# Autodesk Inventor assembly: Transmission
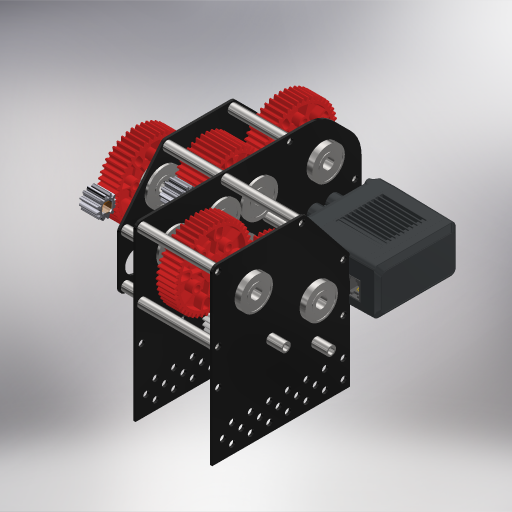
[picture p0: Inventor's stored thumbnail of the model, 512x512]
Saved by Autodesk Inventor 2024 (Build 280153000, 153)
## iProperties
Created: 2023-09-09
Part Number: Transmission
Document SubType Name: Assembly
Designer: aaron
Author: aaron
## Documents named in this file (14)
- C:\Users\aaron\Documents\Inventor\TritonRobotics\library\Stock Material\Plates\POM\Transmision\Transmission.iam
- C:\Users\aaron\Documents\Inventor\TritonRobotics\library\Stock Material\Plates\POM\Transmision\MainLayer.ipt
- C:\Users\aaron\Documents\Inventor\TritonRobotics\library\Stock Material\Plates\POM\Transmision\BottomLayer.ipt
- C:\Users\aaron\Documents\Inventor\TritonRobotics\library\Stock Material\Plates\POM\Transmision\Top Layer.ipt
- C:\Users\aaron\Documents\Inventor\TritonRobotics\library\VEX Library\Structure\Metal Spacers\1.0 1-2 od.ipt
- C:\Users\aaron\Documents\Inventor\TritonRobotics\library\VEX Library\Structure\Metal Spacers\0.25 1-2 od.ipt
- C:\Users\aaron\Documents\Inventor\TritonRobotics\library\VEX Library\Motion\HS Shaft\bearing.ipt
- C:\Users\aaron\Documents\Inventor\TritonRobotics\library\VEX Library\Subsystems\PTOS\PTO .5 v1.1.iam
- C:\Users\aaron\Documents\Inventor\TritonRobotics\library\VEX Library\Subsystems\PTOS\PTO 1 v1.1.iam
- C:\Users\aaron\Documents\Inventor\TritonRobotics\library\VEX Library\Electronics\V5 Motor.ipt
- C:\Users\aaron\Documents\Inventor\TritonRobotics\library\VEX Library\Motion\Gears\High Strength\36 Tooth\36T High Strength Gear v2.ipt
- C:\Users\aaron\Documents\Inventor\TritonRobotics\library\VEX Library\Motion\Gears\Low Strength\36T Gear.ipt
- C:\Users\aaron\Documents\Inventor\TritonRobotics\library\VEX Library\Motion\Gears\High Strength\48 Tooth\48 High Strength Gear V2.ipt
- C:\Users\aaron\Documents\Inventor\TritonRobotics\library\VEX Library\Motion\Gears\High Strength\12 Tooth\HS 12T Gear, No Insert.ipt
## Components (55 placed, 13 different names)
1. MainLayer:1 — Mate:1, Mate:2, Mate:3, Mate:4, Mate:5, Mate:6, Mate:25, Mate:26, Mate:31, Mate:48, Mate:49, Mate:50, Mate:51, Mate:52, Mate:53, Mate:54, Mate:55, Mate:56, Mate:61, Mate:62, Mate:67, Mate:68, Mate:69, Mate:70, Mate:71, Mate:72, Mate:73, Mate:74, Mate:75, Mate:76, Mate:87, Mate:88, Mate:89, Mate:92
2. BottomLayer:1 — Mate:3, Mate:4, Mate:6, Mate:77, Mate:78, Mate:79, Mate:80, Mate:81, Mate:82, Mate:83, Mate:84
3. Top Layer:1 — Mate:1, Mate:2, Mate:5, Mate:9, Mate:10, Mate:17, Mate:18, Mate:19, Mate:20, Mate:21, Mate:22, Mate:63, Mate:64, Mate:65, Mate:66, Mate:85, Mate:86
4. 1.0 1-2 od:1 — Mate:7, Mate:8
5. 1.0 1-2 od:2 — Mate:7, Mate:8, Mate:9, Mate:10
6. 1.0 1-2 od:3 — Mate:17, Mate:18
7. 1.0 1-2 od:4
8. 1.0 1-2 od:5 — Mate:21, Mate:22
9. 1.0 1-2 od:6
10. 1.0 1-2 od:7 — Mate:19, Mate:20
11. 1.0 1-2 od:8
12. 1.0 1-2 od:9 — Mate:26
13. 1.0 1-2 od:10 — Mate:25
14. 1.0 1-2 od:11 — Mate:29, Mate:30
15. 0.25 1-2 od:1 — Mate:27, Mate:28, Mate:29, Mate:30
16. 0.25 1-2 od:2 — Mate:27, Mate:28, Mate:31, Mate:48
17. 1.0 1-2 od:12
18. 0.25 1-2 od:3 — Mate:50
19. 0.25 1-2 od:4 — Mate:49
20. 1.0 1-2 od:13 — Mate:53, Mate:54
21. 0.25 1-2 od:5
22. 0.25 1-2 od:6
23. 1.0 1-2 od:14 — Mate:55, Mate:56
24. 0.25 1-2 od:7
25. 0.25 1-2 od:8
26. 1.0 1-2 od:15 — Mate:51, Mate:52
27. 0.25 1-2 od:9
28. 0.25 1-2 od:10
29. 1.0 1-2 od:16 — Mate:61, Mate:62
30. 0.25 1-2 od:11
31. 0.25 1-2 od:12
32. bearing:1 — Mate:63, Mate:64
33. bearing:2 — Mate:65, Mate:66
34. bearing:3 — Mate:67, Mate:68, Mate:93, Mate:94
35. bearing:4 — Mate:69, Mate:70, Mate:96
36. bearing:5 — Mate:71, Mate:72, Mate:90, Mate:100
37. bearing:6 — Mate:73, Mate:74
38. bearing:7 — Mate:77, Mate:78
39. bearing:8 — Mate:75, Mate:76, Mate:101
40. bearing:9 — Mate:79, Mate:80
41. bearing:10 — Mate:81, Mate:82, Mate:97
42. bearing:11 — Mate:83, Mate:84, Mate:95
43. PTO .5 v1.1:1 [sub-assembly] — Mate:85
44. PTO 1 v1.1:2 [sub-assembly] — Mate:86
45. V5 Motor:1 — Mate:87, Mate:88, Mate:89
46. 36T High Strength Gear v2:1 — Mate:90
47. 36T Gear:1 — Mate:92
48. 48 High Strength Gear V2:1 — Mate:93
49. HS 12T Gear, No Insert:1 — Mate:94
50. 48 High Strength Gear V2:2 — Mate:95
51. HS 12T Gear, No Insert:2 — Mate:96
52. 36T High Strength Gear v2:3 — Mate:97, Mate:98, Mate:99
53. 36T High Strength Gear v2:4 — Mate:98, Mate:99
54. 36T Gear:2 — Mate:100
55. 48 High Strength Gear V2:3 — Mate:101
## Relationships (100: Mate 100)
- Mate:1: MainLayer:1 ↔ Top Layer:1
- Mate:2: MainLayer:1 ↔ Top Layer:1
- Mate:3: MainLayer:1 ↔ BottomLayer:1
- Mate:4: MainLayer:1 ↔ BottomLayer:1
- Mate:5 (50.8 mm): MainLayer:1 ↔ Top Layer:1
- Mate:6 (38.1 mm): MainLayer:1 ↔ BottomLayer:1
- Mate:7: 1.0 1-2 od:1 ↔ 1.0 1-2 od:2
- Mate:8: 1.0 1-2 od:1 ↔ 1.0 1-2 od:2
- Mate:9: Top Layer:1 ↔ 1.0 1-2 od:2
- Mate:10: Top Layer:1 ↔ 1.0 1-2 od:2
- [Mate]: 1.0 1-2 od:3 ↔ 1.0 1-2 od:4
- [Mate]: 1.0 1-2 od:3 ↔ 1.0 1-2 od:4
- [Mate]: 1.0 1-2 od:5 ↔ 1.0 1-2 od:6
- [Mate]: 1.0 1-2 od:5 ↔ 1.0 1-2 od:6
- [Mate]: 1.0 1-2 od:7 ↔ 1.0 1-2 od:8
- [Mate]: 1.0 1-2 od:7 ↔ 1.0 1-2 od:8
- Mate:17: Top Layer:1 ↔ 1.0 1-2 od:3
- Mate:18: Top Layer:1 ↔ 1.0 1-2 od:3
- Mate:19: Top Layer:1 ↔ 1.0 1-2 od:7
- Mate:20: Top Layer:1 ↔ 1.0 1-2 od:7
- Mate:21: Top Layer:1 ↔ 1.0 1-2 od:5
- Mate:22: Top Layer:1 ↔ 1.0 1-2 od:5
- [Mate]: 1.0 1-2 od:9 ↔ 1.0 1-2 od:10
- [Mate]: 1.0 1-2 od:9 ↔ 1.0 1-2 od:10
- Mate:25: MainLayer:1 ↔ 1.0 1-2 od:10
- Mate:26: MainLayer:1 ↔ 1.0 1-2 od:9
- Mate:27: 0.25 1-2 od:1 ↔ 0.25 1-2 od:2
- Mate:28: 0.25 1-2 od:1 ↔ 0.25 1-2 od:2
- Mate:29: 1.0 1-2 od:11 ↔ 0.25 1-2 od:1
- Mate:30: 1.0 1-2 od:11 ↔ 0.25 1-2 od:1
- Mate:31: MainLayer:1 ↔ 0.25 1-2 od:2
- [Mate]: 0.25 1-2 od:3 ↔ 0.25 1-2 od:4
- [Mate]: 0.25 1-2 od:3 ↔ 0.25 1-2 od:4
- [Mate]: 1.0 1-2 od:12 ↔ 0.25 1-2 od:3
- [Mate]: 1.0 1-2 od:12 ↔ 0.25 1-2 od:3
- [Mate]: 0.25 1-2 od:5 ↔ 0.25 1-2 od:6
- [Mate]: 0.25 1-2 od:5 ↔ 0.25 1-2 od:6
- [Mate]: 1.0 1-2 od:13 ↔ 0.25 1-2 od:5
- [Mate]: 1.0 1-2 od:13 ↔ 0.25 1-2 od:5
- [Mate]: 0.25 1-2 od:7 ↔ 0.25 1-2 od:8
- [Mate]: 0.25 1-2 od:7 ↔ 0.25 1-2 od:8
- [Mate]: 1.0 1-2 od:14 ↔ 0.25 1-2 od:7
- [Mate]: 1.0 1-2 od:14 ↔ 0.25 1-2 od:7
- [Mate]: 0.25 1-2 od:9 ↔ 0.25 1-2 od:10
- [Mate]: 0.25 1-2 od:9 ↔ 0.25 1-2 od:10
- [Mate]: 1.0 1-2 od:15 ↔ 0.25 1-2 od:9
- [Mate]: 1.0 1-2 od:15 ↔ 0.25 1-2 od:9
- Mate:48: MainLayer:1 ↔ 0.25 1-2 od:2
- Mate:49: MainLayer:1 ↔ 0.25 1-2 od:4
- Mate:50: MainLayer:1 ↔ 0.25 1-2 od:3
- Mate:51: MainLayer:1 ↔ 1.0 1-2 od:15
- Mate:52: MainLayer:1 ↔ 1.0 1-2 od:15
- Mate:53: MainLayer:1 ↔ 1.0 1-2 od:13
- Mate:54: MainLayer:1 ↔ 1.0 1-2 od:13
- Mate:55: MainLayer:1 ↔ 1.0 1-2 od:14
- Mate:56: MainLayer:1 ↔ 1.0 1-2 od:14
- [Mate]: 0.25 1-2 od:11 ↔ 0.25 1-2 od:12
- [Mate]: 0.25 1-2 od:11 ↔ 0.25 1-2 od:12
- [Mate]: 1.0 1-2 od:16 ↔ 0.25 1-2 od:11
- [Mate]: 1.0 1-2 od:16 ↔ 0.25 1-2 od:11
- Mate:61: MainLayer:1 ↔ 1.0 1-2 od:16
- Mate:62: MainLayer:1 ↔ 1.0 1-2 od:16
- Mate:63: Top Layer:1 ↔ bearing:1
- Mate:64: Top Layer:1 ↔ bearing:1
- Mate:65: Top Layer:1 ↔ bearing:2
- Mate:66: Top Layer:1 ↔ bearing:2
- Mate:67: MainLayer:1 ↔ bearing:3
- Mate:68: MainLayer:1 ↔ bearing:3
- Mate:69: MainLayer:1 ↔ bearing:4
- Mate:70: MainLayer:1 ↔ bearing:4
- Mate:71: MainLayer:1 ↔ bearing:5
- Mate:72: MainLayer:1 ↔ bearing:5
- Mate:73: MainLayer:1 ↔ bearing:6
- Mate:74: MainLayer:1 ↔ bearing:6
- Mate:75: MainLayer:1 ↔ bearing:8
- Mate:76: MainLayer:1 ↔ bearing:8
- Mate:77: BottomLayer:1 ↔ bearing:7
- Mate:78: BottomLayer:1 ↔ bearing:7
- Mate:79: BottomLayer:1 ↔ bearing:9
- Mate:80: BottomLayer:1 ↔ bearing:9
- Mate:81: BottomLayer:1 ↔ bearing:10
- Mate:82: BottomLayer:1 ↔ bearing:10
- Mate:83: BottomLayer:1 ↔ bearing:11
- Mate:84: BottomLayer:1 ↔ bearing:11
- Mate:85: Top Layer:1 ↔ PTO .5 v1.1:1
- Mate:86: Top Layer:1 ↔ PTO 1 v1.1:2
- Mate:87: MainLayer:1 ↔ V5 Motor:1
- Mate:88: MainLayer:1 ↔ V5 Motor:1
- Mate:89: MainLayer:1 ↔ V5 Motor:1
- Mate:90: bearing:5 ↔ 36T High Strength Gear v2:1
- Mate:92: MainLayer:1 ↔ 36T Gear:1
- Mate:93: bearing:3 ↔ 48 High Strength Gear V2:1
- Mate:94: bearing:3 ↔ HS 12T Gear, No Insert:1
- Mate:95: bearing:11 ↔ 48 High Strength Gear V2:2
- Mate:96: bearing:4 ↔ HS 12T Gear, No Insert:2
- Mate:97: bearing:10 ↔ 36T High Strength Gear v2:3
- Mate:98: 36T High Strength Gear v2:3 ↔ 36T High Strength Gear v2:4
- Mate:99: 36T High Strength Gear v2:3 ↔ 36T High Strength Gear v2:4
- Mate:100: bearing:5 ↔ 36T Gear:2
- Mate:101: bearing:8 ↔ 48 High Strength Gear V2:3
## Named parameters: d16_d12 = 0 mm, d17_d13 = 0 mm, d18_d12 = 0 mm, d19_d13 = 0 mm, d20_d12 = 0 mm, d21_d13 = 0 mm, d28_d12 = 0 mm, d29_d13 = 0 mm, d37_d32 = 0 mm, d38_d33 = 0 mm, d39_d34 = 0 mm, d40_d35 = 0 mm, d41_d32 = 0 mm, d42_d33 = 0 mm, d43_d34 = 0 mm, d44_d35 = 0 mm, d45_d32 = 0 mm, d46_d33 = 0 mm, d47_d34 = 0 mm, d48_d35 = 0 mm, d49_d32 = 0 mm, d50_d33 = 0 mm, d51_d34 = 0 mm, d52_d35 = 0 mm, d62_d32 = 0 mm, d63_d33 = 0 mm, d64_d34 = 0 mm, d65_d35 = 0 mm
